# Autodesk Inventor assembly: S8x4
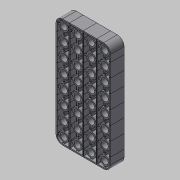
[picture p0: Inventor's stored thumbnail of the model, 180x180]
Saved by Autodesk Inventor 2020 (Build 240168000, 168)
## iProperties
Created: 2019-04-29
Part Number: S8x4
Document SubType Name: Assembly
Designer: Varga Daniel
Author: Varga Daniel
## Documents named in this file (6)
- C:\!_Dani\!_cloud\OneDrive\!_munka\Revolution\StructuralParts\Beams\Straight Beams\S3+x3+\S8x4.iam
- C:\!_Dani\!_cloud\OneDrive\!_munka\Revolution\StructuralParts\Beams\beam_corner_part.ipt
- C:\!_Dani\!_cloud\OneDrive\!_munka\Revolution\StructuralParts\Beams\beam_side_part.ipt
- C:\!_Dani\!_cloud\OneDrive\!_munka\Revolution\StructuralParts\Beams\beam_top_bot_part.ipt
- C:\!_Dani\!_cloud\OneDrive\!_munka\Revolution\StructuralParts\Beams\beam_inner_part.ipt
- C:\!_Dani\!_cloud\OneDrive\!_munka\Revolution\StructuralParts\Beams\Straight Beams\S3+x3+.iam
## Components (32 placed, 4 different names)
1. beam_corner_part:1 — Flush:1, Flush:2, Flush:3, Flush:4, Flush:5, Mate:4, Flush:6, Flush:7, Width_displacement, Flush:12, Mate:6, Flush:13, Flush:14, Flush:15
2. beam_corner_part:2 — Length_displacement, Flush:6, Flush:7, Width_displacement
3. beam_corner_part:3 — Flush:16, Flush:17, Mate:10
4. beam_corner_part:4 — Length_displacement, Flush:14, Flush:15, Flush:16, Flush:17, Flush:18, Flush:19, Mate:9, Mate:10
5. beam_top_bot_part:1 — Flush:4, Flush:5, Mate:4
6. beam_top_bot_part:3
7. beam_side_part:1 — Flush:8, Flush:9, Flush:10, Flush:11, Flush:12, Mate:6, Mate:7, Flush:13, Mate:8
8. beam_side_part:2 — Flush:10, Flush:11, Mate:8
9. beam_side_part:3
10. beam_side_part:4
11. beam_side_part:5
12. beam_side_part:6
13. beam_side_part:7
14. beam_side_part:8
15. beam_side_part:9
16. beam_side_part:10
17. beam_side_part:11
18. beam_side_part:12
19. beam_top_bot_part:2 — Flush:18, Flush:19, Mate:9
20. beam_top_bot_part:4
21. beam_inner_part:1 — Flush:8, Flush:9, Mate:7
22. beam_inner_part:4
23. beam_inner_part:3
24. beam_inner_part:5
25. beam_inner_part:6
26. beam_inner_part:7
27. beam_inner_part:8
28. beam_inner_part:9
29. beam_inner_part:10
30. beam_inner_part:11
31. beam_inner_part:12
32. beam_inner_part:13
## Component patterns: (2 elements, first: beam_top_bot_part:1), (6 elements, first: beam_side_part:1 + beam_side_part:2), (2 elements, first: beam_top_bot_part:2), (2 elements, first: beam_inner_part:1), Component Pattern 4:2 (2 elements), Component Pattern 4:3 (2 elements), Component Pattern 4:4 (2 elements), Component Pattern 4:5 (2 elements), Component Pattern 4:6 (2 elements)
## Relationships (27: Flush 19, Mate 8)
- Flush:1: beam_corner_part:1
- Flush:2: beam_corner_part:1
- Flush:3: beam_corner_part:1
- Length_displacement [Mate] (60 mm): beam_corner_part:2 ↔ beam_corner_part:4
- Flush:4: beam_corner_part:1 ↔ beam_top_bot_part:1
- Flush:5: beam_corner_part:1 ↔ beam_top_bot_part:1
- Mate:4: beam_corner_part:1 ↔ beam_top_bot_part:1
- Flush:6: beam_corner_part:1 ↔ beam_corner_part:2
- Flush:7: beam_corner_part:1 ↔ beam_corner_part:2
- Width_displacement [Mate] (20 mm): beam_corner_part:1 ↔ beam_corner_part:2
- Flush:8: beam_side_part:1 ↔ beam_inner_part:1
- Flush:9: beam_side_part:1 ↔ beam_inner_part:1
- Flush:10: beam_side_part:1 ↔ beam_side_part:2
- Flush:11: beam_side_part:1 ↔ beam_side_part:2
- Flush:12: beam_corner_part:1 ↔ beam_side_part:1
- Mate:6: beam_corner_part:1 ↔ beam_side_part:1
- Mate:7: beam_side_part:1 ↔ beam_inner_part:1
- Flush:13: beam_corner_part:1 ↔ beam_side_part:1
- Mate:8 (20 mm): beam_side_part:1 ↔ beam_side_part:2
- Flush:14: beam_corner_part:1 ↔ beam_corner_part:4
- Flush:15: beam_corner_part:1 ↔ beam_corner_part:4
- Flush:16: beam_corner_part:3 ↔ beam_corner_part:4
- Flush:17: beam_corner_part:3 ↔ beam_corner_part:4
- Flush:18: beam_corner_part:4 ↔ beam_top_bot_part:2
- Flush:19: beam_corner_part:4 ↔ beam_top_bot_part:2
- Mate:9: beam_corner_part:4 ↔ beam_top_bot_part:2
- Mate:10 (20 mm): beam_corner_part:3 ↔ beam_corner_part:4
